# Autodesk Inventor assembly: camera_mount
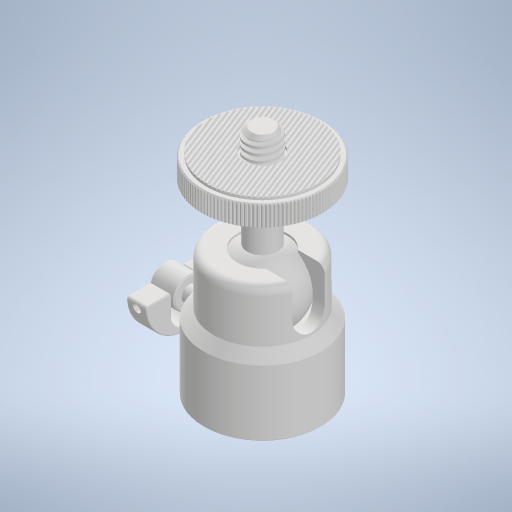
[picture p0: Inventor's stored thumbnail of the model, 512x512]
Saved by Autodesk Inventor 2023 (Build 270158000, 158)
## iProperties
Created: 2011-12-13
Part Number: camera_mount
Description: STEP AP203
Document SubType Name: Assembly
Designer: Robert
Sending System: SolidWorks 2011
Preprocessor: SwSTEP 2.0
Title: Main Assembly.STEP
Revision Number: ANY
## Documents named in this file (11)
- C:\Users\Rober\Documents\Ingenieurinformatik\grop\catkin\src\grop\robot_gripper_camera\meshes\camera_mount.iam
- C:\Users\Rober\Documents\Ingenieurinformatik\grop\catkin\src\grop\robot_gripper_camera\meshes\Circlip.ipt
- C:\Users\Rober\Documents\Ingenieurinformatik\grop\catkin\src\grop\robot_gripper_camera\meshes\Locking Screw Pin.ipt
- C:\Users\Rober\Documents\Ingenieurinformatik\grop\catkin\src\grop\robot_gripper_camera\meshes\Anti-Slip Pad.ipt
- C:\Users\Rober\Documents\Ingenieurinformatik\grop\catkin\src\grop\robot_gripper_camera\meshes\Anchor Plate.ipt
- C:\Users\Rober\Documents\Ingenieurinformatik\grop\catkin\src\grop\robot_gripper_camera\meshes\Swivel Body.ipt
- C:\Users\Rober\Documents\Ingenieurinformatik\grop\catkin\src\grop\robot_gripper_camera\meshes\Swivel Lock Seat.ipt
- C:\Users\Rober\Documents\Ingenieurinformatik\grop\catkin\src\grop\robot_gripper_camera\meshes\Lock Nut.ipt
- C:\Users\Rober\Documents\Ingenieurinformatik\grop\catkin\src\grop\robot_gripper_camera\meshes\Locking Screw.ipt
- C:\Users\Rober\Documents\Ingenieurinformatik\grop\catkin\src\grop\robot_gripper_camera\meshes\Swivel.ipt
- C:\Users\Rober\Documents\Ingenieurinformatik\grop\catkin\src\grop\robot_gripper_camera\meshes\Locking Screw Handle.ipt
## Components (10 placed, 10 different names)
1. Circlip_2 — Passend:10, Winkel:4, Passend:11, Passend:12
2. Locking Screw Pin_4 — Passend:4, Passend:6
3. Anti-Slip Pad_6 — Einfügen:2
4. Anchor Plate_9 — Passend:8, Winkel:3, Passend:12
5. Swivel Body_10 — Passend:1, Passend:2, Winkel:1, Tangential:1, Passend:3, Passend:8, Passend:10, Passend:11, Winkel:5, Winkel:6
6. Swivel Lock Seat_14 — Tangential:2, Winkel:2, Tangential:3
7. Lock Nut_16 — Einfügen:1, Einfügen:2, Winkel:6
8. Locking Screw_17 — Passend:3, Tangential:3, Passend:5, Passend:6, Passend:7, Winkel:3, Winkel:4
9. Swivel_18 — Einfügen:1, Tangential:1, Tangential:2
10. Locking Screw Handle_23 — Passend:4, Passend:5, Passend:7, Winkel:5
## Relationships (22: Mate 11, Angle 6, Tangent 3, Insert 2)
- Passend:1 [Mate]: Swivel Body_10
- Passend:2 [Mate]: Swivel Body_10
- Winkel:1 [Angle] (0 deg): Swivel Body_10
- Einfügen:1 [Insert]: Lock Nut_16 ↔ Swivel_18
- Einfügen:2 [Insert]: Anti-Slip Pad_6 ↔ Lock Nut_16
- Tangential:1: Swivel Body_10 ↔ Swivel_18
- Tangential:2: Swivel Lock Seat_14 ↔ Swivel_18
- Winkel:2 [Angle] (0 deg): Swivel Lock Seat_14
- Passend:3 [Mate]: Swivel Body_10 ↔ Locking Screw_17
- Tangential:3: Swivel Lock Seat_14 ↔ Locking Screw_17
- Passend:4 [Mate]: Locking Screw Pin_4 ↔ Locking Screw Handle_23
- Passend:5 [Mate]: Locking Screw_17 ↔ Locking Screw Handle_23
- Passend:6 [Mate]: Locking Screw Pin_4 ↔ Locking Screw_17
- Passend:7 [Mate]: Locking Screw_17 ↔ Locking Screw Handle_23
- Passend:8 [Mate]: Anchor Plate_9 ↔ Swivel Body_10
- Winkel:3 [Angle] (0 deg): Anchor Plate_9 ↔ Locking Screw_17
- Passend:10 [Mate]: Circlip_2 ↔ Swivel Body_10
- Winkel:4 [Angle] (0 deg): Circlip_2 ↔ Locking Screw_17
- Passend:11 [Mate]: Circlip_2 ↔ Swivel Body_10
- Passend:12 [Mate]: Circlip_2 ↔ Anchor Plate_9
- Winkel:5 [Angle] (0 deg): Swivel Body_10 ↔ Locking Screw Handle_23
- Winkel:6 [Angle] (0 deg): Swivel Body_10 ↔ Lock Nut_16
